# Autodesk Inventor assembly: PSCTW10
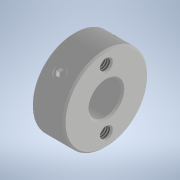
[picture p0: Inventor's stored thumbnail of the model, 180x180]
Saved by Autodesk Inventor 2021 (Build 250183000, 183)
## iProperties
Category: PARTsolutions
Company: MISUMI
Created: 2025-04-29
Part Number: PSCTW10
Catalog Web Link: www.cadenas.de
Description: SCTW, PSCTW, SSCTW-Shaft Collars - Set Screw, with 2 Holes
Vendor: MISUMI
Document SubType Name: Assembly
Designer: psAdmin
Manufacturer: MISUMI
Mass: 4.27292 g
Surface Area: 24.1107 cm^2
Volume: 4.27292 cm^3
Density: 1 g/cm^3
Title: PSCTW10
Author: Cadenas PARTsolutions
Comments: Shaft Collars - Set Screw, with 2 Holes
PSOL_IDENT_0: {$CADENAS_DATA/23d-libs/misumi/metric/03_set_collars/sctw_asmtab.prj},186 {VTYP=3D},{STYP=ASSTAB},{N
PSOL_IDENT_1: B=PSCTW10},{LINA=PSCTW10},{NN=SCTW, PSCTW, SSCTW},{DATE=02.06.2021 03:00:04},{GEOMDATE=25.12.2015 07
PSOL_IDENT_2: :49:56},{VERSION=},{LINEID=60},{WBVAR=MAT,ST},{WBNUMERIC=}  {NB=PSCTW10},{LINA=PSCTW10},{KT=DUMMY},{
PSOL_IDENT_3: PN=PSCTW10},{TYPE=PSCTW},{MAT=1045},{ST=Electroless Nickel Plating},{AC=Set Screws 2 Pcs. (304 Stain
PSOL_IDENT_4: less Steel) },{D=10},{B=10},{D1=26},{P=18},{M=M4x4},{THMD=4},{THDMIN=3.242},{M1=M4},{C=0.5},{ST0='Bl
PSOL_IDENT_5: ack Oxide','Black Oxide','Electroless Nickel Plating','Electroless Nickel Plating'},{L=4},{PPATH=sct
PSOL_IDENT_6: w/sctw_asmtpl.prj}
NB: PSCTW10
NN: SCTW, PSCTW, SSCTW
NT: Shaft Collars - Set Screw, with 2 Holes
NBSYN: $PN.
LINA: PSCTW10
CATALOG: Misumi
PN: PSCTW10
MAT: S45C Equivalent
ST: Electroless Nickel Plating
AC: Set Screws 2 Pcs. (304 Stainless Steel)
D: 10
B: 10
D1: 26
P: 18
M: M4x4
M1: M4
SUPPLIER: MISUMI
ARTICLENO: PSCTW10
BOMINFO: PSCTW10
CREATOR: CADENAS GmbH
## Documents named in this file (3)
- e:\temp\worker_COMMON_350\temp\tmp_8240_214_MshEY\format_0\PSCTW10.iam
- e:\temp\worker_COMMON_350\temp\tmp_8240_214_MshEY\format_0\PSCTW10b.ipt
- e:\temp\worker_COMMON_350\temp\tmp_8240_214_MshEY\format_0\Hexagon socket set screw with flat point DIN 913 - M4x4.ipt
## Components (3 placed, 2 different names)
1. PSCTW10b:1 — body_set_v_XY@1 <-> IP1_XY@2, body_set_v_Z@1 <-> IP1_Z@2, body_set_v_YZ@1 <-> IP1_YZ@2, body_set_h_XY@1 <-> IP1_XY@3, body_set_h_Z@1 <-> IP1_Z@3, body_set_h_YZ@1 <-> IP1_YZ@3
2. Hexagon socket set screw with flat point DIN 913 - M4x4:1 — body_set_v_XY@1 <-> IP1_XY@2, body_set_v_Z@1 <-> IP1_Z@2, body_set_v_YZ@1 <-> IP1_YZ@2
3. Hexagon socket set screw with flat point DIN 913 - M4x4:2 — body_set_h_XY@1 <-> IP1_XY@3, body_set_h_Z@1 <-> IP1_Z@3, body_set_h_YZ@1 <-> IP1_YZ@3
## Relationships (6: Mate 3, Angle 2, Flush 1)
- body_set_v_XY@1 <-> IP1_XY@2 [Mate]: PSCTW10b:1 ↔ Hexagon socket set screw with flat point DIN 913 - M4x4:1
- body_set_v_Z@1 <-> IP1_Z@2 [Mate]: PSCTW10b:1 ↔ Hexagon socket set screw with flat point DIN 913 - M4x4:1
- body_set_v_YZ@1 <-> IP1_YZ@2 [Angle] (0 deg): PSCTW10b:1 ↔ Hexagon socket set screw with flat point DIN 913 - M4x4:1
- body_set_h_XY@1 <-> IP1_XY@3 [Flush]: PSCTW10b:1 ↔ Hexagon socket set screw with flat point DIN 913 - M4x4:2
- body_set_h_Z@1 <-> IP1_Z@3 [Mate]: PSCTW10b:1 ↔ Hexagon socket set screw with flat point DIN 913 - M4x4:2
- body_set_h_YZ@1 <-> IP1_YZ@3 [Angle] (0 deg): PSCTW10b:1 ↔ Hexagon socket set screw with flat point DIN 913 - M4x4:2
